# Autodesk Inventor assembly: AssemblyAnalysis
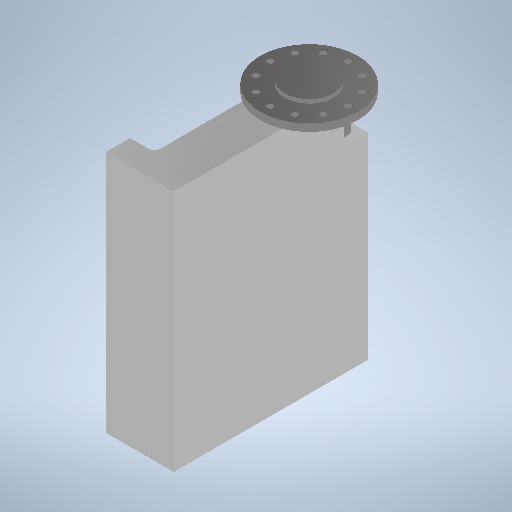
[picture p0: Inventor's stored thumbnail of the model, 512x512]
Saved by Autodesk Inventor 2025.1 (Build 291241000, 241)
## iProperties
Created: 2025-01-29
Part Number: AssemblyAnalysis
Document SubType Name: Assembly
Designer: yovan
Author: yovan
## Documents named in this file (9)
- C:\Users\yovan\Desktop\APM\ausol-apm.github.io\project\Design and simulation\Inventor\CeldaRobótica1\AssemblyAnalysis.iam
- C:\Users\yovan\Desktop\APM\ausol-apm.github.io\project\Design and simulation\Inventor\CeldaRobótica1\EndEffector.ipt
- C:\Users\yovan\Desktop\APM\ausol-apm.github.io\project\Design and simulation\Inventor\CeldaRobótica1\MoldeR.ipt
- C:\Users\yovan\Desktop\APM\ausol-apm.github.io\project\Design and simulation\Inventor\CeldaRobótica1\AssemblyAnalysis\AIP\FEA\eyi5mwx6o.fins
- C:\Users\yovan\Desktop\APM\ausol-apm.github.io\project\Design and simulation\Inventor\CeldaRobótica1\AssemblyAnalysis\AIP\FEA\eyi5mwx6o.fsat
- C:\Users\yovan\Desktop\APM\ausol-apm.github.io\project\Design and simulation\Inventor\CeldaRobótica1\AssemblyAnalysis\AIP\FEA\eyi5mwx6o.ftes
- C:\Users\yovan\Desktop\APM\ausol-apm.github.io\project\Design and simulation\Inventor\CeldaRobótica1\AssemblyAnalysis\AIP\FEA\eyi5mwx6o.fwiz
- C:\Users\yovan\Desktop\APM\ausol-apm.github.io\project\Design and simulation\Inventor\CeldaRobótica1\AssemblyAnalysis\AIP\FEA\eyi5mwx7k.fmsh
- C:\Users\yovan\Desktop\APM\ausol-apm.github.io\project\Design and simulation\Inventor\CeldaRobótica1\AssemblyAnalysis\AIP\FEA\eyi5mwx8g.fres
## Components (2 placed, 2 different names)
1. EndEffector:1 — Insert:1, Insert:2
2. MoldeR:1 — Insert:1, Insert:2
## Relationships (2: Insert 2)
- Insert:1: EndEffector:1 ↔ MoldeR:1
- Insert:2: EndEffector:1 ↔ MoldeR:1
